# Autodesk Inventor assembly: termoformadora
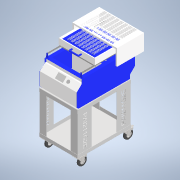
[picture p0: Inventor's stored thumbnail of the model, 180x180]
Saved by Autodesk Inventor 2021 (Build 250183000, 183)
## iProperties
Created: 2021-04-15
Part Number: termoformadora
Document SubType Name: Assembly
Designer: Leonardo Fabio Mercado Benítez
Author: Leonardo Fabio Mercado Benítez
## Documents named in this file (13)
- C:\Users\Nelson\Github\Proyecto_PAI_2021\01 CAD\termoformadora.iam
- C:\Users\Nelson\Github\Proyecto_PAI_2021\01 CAD\Ensamblaje carcasa superior.iam
- C:\Users\Nelson\Github\Proyecto_PAI_2021\01 CAD\soporte_inferior_zona_calor.ipt
- C:\Users\Nelson\Github\Proyecto_PAI_2021\01 CAD\tapa_caja_calor.ipt
- C:\Users\Nelson\Github\Proyecto_PAI_2021\01 CAD\angulo_caja_calor.ipt
- C:\Users\Nelson\Github\Proyecto_PAI_2021\01 CAD\buje_carro_zona_calor.ipt
- C:\Users\Nelson\Github\Proyecto_PAI_2021\01 CAD\barra.ipt
- C:\Users\Nelson\Github\Proyecto_PAI_2021\01 CAD\mango_zona_calor.ipt
- C:\Users\Nelson\Github\Proyecto_PAI_2021\01 CAD\Ensamblaje carcasa control.iam
- C:\Users\Nelson\Github\Proyecto_PAI_2021\01 CAD\soporte_barra.ipt
- C:\Users\Nelson\Github\Proyecto_PAI_2021\01 CAD\ensamble resistencias.iam
- C:\Users\Nelson\Github\Proyecto_PAI_2021\01 CAD\soporte_resistencias.ipt
- C:\Users\Nelson\Github\Proyecto_PAI_2021\01 CAD\Estructura Lámina.iam
## Components (18 placed, 12 different names)
1. Ensamblaje carcasa superior:1 [sub-assembly] — Coincidencia:1, Coincidencia:2, Coincidencia:11, Coincidencia:12, Nivelación:7, Coincidencia:16, Coincidencia:17
2. soporte_inferior_zona_calor:1 — Coincidencia:1, Coincidencia:2, Coincidencia:3, Nivelación:1, Nivelación:2, Coincidencia:5, Nivelación:3, Nivelación:4, Coincidencia:6, Nivelación:5, Nivelación:6, Coincidencia:15, Insertar:5, Insertar:6, Coincidencia:27, Coincidencia:28, Coincidencia:30
3. tapa_caja_calor:1 — Coincidencia:3, Nivelación:1, Nivelación:2
4. angulo_caja_calor:1 — Coincidencia:5, Nivelación:3, Nivelación:4, Coincidencia:7, Coincidencia:8, Insertar:1, Insertar:2
5. angulo_caja_calor:2 — Coincidencia:6, Nivelación:5, Nivelación:6, Coincidencia:9, Coincidencia:10, Insertar:3, Insertar:4
6. buje_carro_zona_calor:1 — Coincidencia:9, Insertar:3
7. buje_carro_zona_calor:2 — Coincidencia:8, Insertar:2, Coincidencia:14
8. buje_carro_zona_calor:3 — Coincidencia:10, Insertar:4
9. buje_carro_zona_calor:4 — Coincidencia:7, Insertar:1, Coincidencia:13
10. barra:1 — Coincidencia:11, Coincidencia:13, Coincidencia:21
11. barra:2 — Coincidencia:12, Coincidencia:14, Coincidencia:22
12. mango_zona_calor:1 — Coincidencia:15, Insertar:5, Insertar:6
13. Ensamblaje carcasa control:1 [sub-assembly] — Nivelación:7, Coincidencia:16, Coincidencia:17, Nivelación:8, Coincidencia:18, Coincidencia:20, Nivelación:9, Coincidencia:23, Coincidencia:33, Nivelación:10, Nivelación:11
14. soporte_barra:1 — Nivelación:8, Coincidencia:18, Coincidencia:22
15. soporte_barra:2 — Coincidencia:20, Nivelación:9, Coincidencia:21
16. ensamble resistencias:1 [sub-assembly] — Coincidencia:23, Coincidencia:29, Coincidencia:31, Coincidencia:32
17. soporte_resistencias:1 — Coincidencia:27, Coincidencia:28, Coincidencia:29, Coincidencia:30, Coincidencia:31, Coincidencia:32
18. Estructura Lámina:1 [sub-assembly] — Coincidencia:33, Nivelación:10, Nivelación:11
## Relationships (45: Mate 28, Flush 11, Insert 6)
- Coincidencia:1 [Mate] (61.24 mm): Ensamblaje carcasa superior:1 ↔ soporte_inferior_zona_calor:1
- Coincidencia:2 [Mate] (29 mm): Ensamblaje carcasa superior:1 ↔ soporte_inferior_zona_calor:1
- Coincidencia:3 [Mate]: soporte_inferior_zona_calor:1 ↔ tapa_caja_calor:1
- Nivelación:1 [Flush] (12.7 mm): soporte_inferior_zona_calor:1 ↔ tapa_caja_calor:1
- Nivelación:2 [Flush] (12.7 mm): soporte_inferior_zona_calor:1 ↔ tapa_caja_calor:1
- Coincidencia:5 [Mate]: soporte_inferior_zona_calor:1 ↔ angulo_caja_calor:1
- Nivelación:3 [Flush]: soporte_inferior_zona_calor:1 ↔ angulo_caja_calor:1
- Nivelación:4 [Flush] (10 mm): soporte_inferior_zona_calor:1 ↔ angulo_caja_calor:1
- Coincidencia:6 [Mate]: soporte_inferior_zona_calor:1 ↔ angulo_caja_calor:2
- Nivelación:5 [Flush]: soporte_inferior_zona_calor:1 ↔ angulo_caja_calor:2
- Nivelación:6 [Flush]: soporte_inferior_zona_calor:1 ↔ angulo_caja_calor:2
- Coincidencia:7 [Mate]: angulo_caja_calor:1 ↔ buje_carro_zona_calor:4
- Coincidencia:8 [Mate]: angulo_caja_calor:1 ↔ buje_carro_zona_calor:2
- Coincidencia:9 [Mate]: angulo_caja_calor:2 ↔ buje_carro_zona_calor:1
- Coincidencia:10 [Mate]: angulo_caja_calor:2 ↔ buje_carro_zona_calor:3
- Insertar:1: angulo_caja_calor:1 ↔ buje_carro_zona_calor:4
- Insertar:2: angulo_caja_calor:1 ↔ buje_carro_zona_calor:2
- Insertar:3: angulo_caja_calor:2 ↔ buje_carro_zona_calor:1
- Insertar:4: angulo_caja_calor:2 ↔ buje_carro_zona_calor:3
- Coincidencia:11 [Mate]: Ensamblaje carcasa superior:1 ↔ barra:1
- Coincidencia:12 [Mate]: Ensamblaje carcasa superior:1 ↔ barra:2
- Coincidencia:13 [Mate]: buje_carro_zona_calor:4 ↔ barra:1
- Coincidencia:14 [Mate]: buje_carro_zona_calor:2 ↔ barra:2
- Coincidencia:15 [Mate]: soporte_inferior_zona_calor:1 ↔ mango_zona_calor:1
- Insertar:5: soporte_inferior_zona_calor:1 ↔ mango_zona_calor:1
- Insertar:6: soporte_inferior_zona_calor:1 ↔ mango_zona_calor:1
- Nivelación:7 [Flush] (-74.1 mm): Ensamblaje carcasa superior:1 ↔ Ensamblaje carcasa control:1
- Coincidencia:16 [Mate] (-43.5 mm): Ensamblaje carcasa superior:1 ↔ Ensamblaje carcasa control:1
- Coincidencia:17 [Mate] (53.74 mm): Ensamblaje carcasa superior:1 ↔ Ensamblaje carcasa control:1
- Nivelación:8 [Flush] (5 mm): Ensamblaje carcasa control:1 ↔ soporte_barra:1
- Coincidencia:18 [Mate]: Ensamblaje carcasa control:1 ↔ soporte_barra:1
- Coincidencia:20 [Mate]: Ensamblaje carcasa control:1 ↔ soporte_barra:2
- Nivelación:9 [Flush] (5 mm): Ensamblaje carcasa control:1 ↔ soporte_barra:2
- Coincidencia:21 [Mate]: barra:1 ↔ soporte_barra:2
- Coincidencia:22 [Mate]: barra:2 ↔ soporte_barra:1
- Coincidencia:23 [Mate] (106 mm): Ensamblaje carcasa control:1 ↔ ensamble resistencias:1
- Coincidencia:27 [Mate] (0.5 mm): soporte_inferior_zona_calor:1 ↔ soporte_resistencias:1
- Coincidencia:28 [Mate] (0.5 mm): soporte_inferior_zona_calor:1 ↔ soporte_resistencias:1
- Coincidencia:29 [Mate]: ensamble resistencias:1 ↔ soporte_resistencias:1
- Coincidencia:30 [Mate] (59.36 mm): soporte_inferior_zona_calor:1 ↔ soporte_resistencias:1
- Coincidencia:31 [Mate] (31.54 mm): ensamble resistencias:1 ↔ soporte_resistencias:1
- Coincidencia:32 [Mate] (32.2 mm): ensamble resistencias:1 ↔ soporte_resistencias:1
- Coincidencia:33 [Mate]: Ensamblaje carcasa control:1 ↔ Estructura Lámina:1
- Nivelación:10 [Flush] (10 mm): Ensamblaje carcasa control:1 ↔ Estructura Lámina:1
- Nivelación:11 [Flush]: Ensamblaje carcasa control:1 ↔ Estructura Lámina:1
